# Autodesk Inventor assembly: Elevator
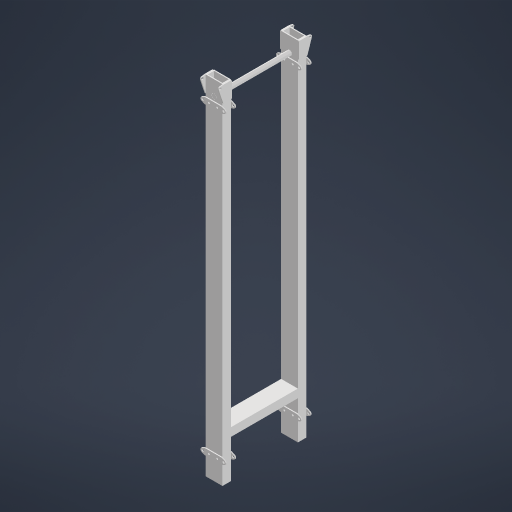
[picture p0: Inventor's stored thumbnail of the model, 512x512]
Saved by Autodesk Inventor 2023 (Build 270158000, 158)
## iProperties
Created: 2023-01-15
Part Number: Elevator
Document SubType Name: Assembly
Designer: Terrence
Mass: 2162.29 g
Surface Area: 5804.92 cm^2
Volume: 800.848 cm^3
Density: 2.7 g/cm^3
Author: Terrence
## Documents named in this file (8)
- C:\Users\Terrence\Documents\FRC Long\Newvator\Elevator.iam
- C:\Users\Terrence\Documents\FRC Long\Newvator\Solid1_1.ipt
- C:\Users\Terrence\Documents\FRC Long\Newvator\Solid2_1.ipt
- C:\Users\Terrence\Documents\FRC Long\Newvator\Solid3_1.ipt
- C:\Users\Terrence\Documents\FRC Long\Newvator\Solid4_1.ipt
- C:\Users\Terrence\Documents\FRC Long\Newvator\Solid5.ipt
- C:\Users\Terrence\Documents\FRC Long\Newvator\Solid7.ipt
- C:\Users\Terrence\Documents\FRC Long\Newvator\Solid9.ipt
## Components (21 placed, 7 different names)
1. Solid1_1:1 — Insert:5, Insert:6, Insert:21, Insert:22, Insert:25, Insert:26, Insert:31, Insert:32
2. Solid2_1:1
3. Solid3_1:1
4. Solid4_1:1
5. Solid5:1
6. Solid1_1:2 — Insert:17, Insert:18, Insert:19, Insert:20, Insert:23, Insert:24, Insert:27, Insert:28, Insert:29, Insert:30
7. Solid5:2
8. Solid4_1:2 — Insert:5, Insert:6
9. Solid4_1:3 — Insert:17, Insert:18
10. Solid4_1:4 — Insert:19, Insert:20
11. Solid3_1:2 — Insert:31, Insert:32
12. Solid3_1:3
13. Solid5:3
14. Solid5:5
15. Solid3_1:8 — Insert:21, Insert:22
16. Solid3_1:9 — Insert:23, Insert:24
17. Solid3_1:10 — Insert:25, Insert:26
18. Solid3_1:11 — Insert:27, Insert:28
19. Solid3_1:12 — Insert:29, Insert:30
20. Solid7:1
21. Solid9:1
## Relationships (18: Insert 18)
- Insert:5: Solid1_1:1 ↔ Solid4_1:2
- Insert:6: Solid1_1:1 ↔ Solid4_1:2
- Insert:17: Solid1_1:2 ↔ Solid4_1:3
- Insert:18: Solid1_1:2 ↔ Solid4_1:3
- Insert:19: Solid1_1:2 ↔ Solid4_1:4
- Insert:20: Solid1_1:2 ↔ Solid4_1:4
- Insert:21: Solid1_1:1 ↔ Solid3_1:8
- Insert:22: Solid1_1:1 ↔ Solid3_1:8
- Insert:23: Solid1_1:2 ↔ Solid3_1:9
- Insert:24: Solid1_1:2 ↔ Solid3_1:9
- Insert:25: Solid1_1:1 ↔ Solid3_1:10
- Insert:26: Solid1_1:1 ↔ Solid3_1:10
- Insert:27: Solid1_1:2 ↔ Solid3_1:11
- Insert:28: Solid1_1:2 ↔ Solid3_1:11
- Insert:29: Solid1_1:2 ↔ Solid3_1:12
- Insert:30: Solid1_1:2 ↔ Solid3_1:12
- Insert:31: Solid1_1:1 ↔ Solid3_1:2
- Insert:32: Solid1_1:1 ↔ Solid3_1:2
